# Autodesk Inventor assembly: wheel_dual
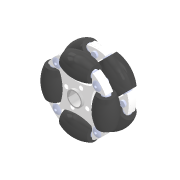
[picture p0: Inventor's stored thumbnail of the model, 180x180]
Saved by Autodesk Inventor 2020 (Build 240168000, 168)
## iProperties
Created: 2019-11-04
Part Number: wheel_dual
Document SubType Name: Assembly
Designer: ball
Author: ball
## Documents named in this file (3)
- C:\FTC\FTC8863CAD\2019 Robot\Odoemetry module\wheel_dual.iam
- C:\FTC\FTC8863CAD\2019 Robot\Odoemetry module\wheel single.iam
- C:\FTC\FTC8863CAD\2019 Robot\Odoemetry module\Our omiwheelinsert.ipt
## Components (3 placed, 2 different names)
1. wheel single:1 [sub-assembly] — Mate:1, Mate:2, Mate:3, Mate:5
2. wheel single:2 [sub-assembly] — Mate:4, Mate:5, Mate:6
3. Our omiwheelinsert:1 — Mate:1, Mate:2, Mate:3, Mate:4, Mate:6
## Relationships (6: Mate 6)
- Mate:1: wheel single:1 ↔ Our omiwheelinsert:1
- Mate:2: wheel single:1 ↔ Our omiwheelinsert:1
- Mate:3: wheel single:1 ↔ Our omiwheelinsert:1
- Mate:4: wheel single:2 ↔ Our omiwheelinsert:1
- Mate:5: wheel single:1 ↔ wheel single:2
- Mate:6: wheel single:2 ↔ Our omiwheelinsert:1
